# Autodesk Inventor assembly: Y_Axes
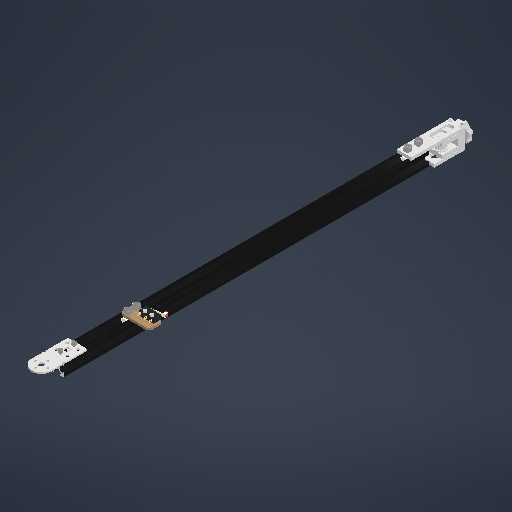
[picture p0: Inventor's stored thumbnail of the model, 512x512]
Saved by Autodesk Inventor 2027.1 (Build 311270010, 270A)
## iProperties
Created: 2026-10-02
Part Number: Y_Axes
Document SubType Name: Assembly
Designer: SDS Scholar
Author: SDS Scholar
## Documents named in this file (13)
- E:\Apps\AutodeskInventor\University\MCT333_Design_of_Mechatronics_Systems_1\CAD\cartesian_robot_workspace\Y_Axis.iam
- E:\Apps\AutodeskInventor\University\MCT333_Design_of_Mechatronics_Systems_1\CAD\off_the_shelf_components\AluminiumExtrusion\AluminiumExtrusion2020\Y_axis.ipt
- E:\Apps\AutodeskInventor\University\MCT333_Design_of_Mechatronics_Systems_1\CAD\off_the_shelf_components\GT2BeltTensioner\2020 Belt Tensioner G_K.ipt
- E:\Apps\AutodeskInventor\University\MCT333_Design_of_Mechatronics_Systems_1\CAD\off_the_shelf_components\T_nuts\Slider T-Nut for 2020 - M5.ipt
- C:\Users\SDS Scholar\Documents\Inventor\Content Center Files\R2027\en-US\SS-ISO 4762\ISO 4762 - M5 x 12SS-ISO.ipt
- E:\Apps\AutodeskInventor\University\MCT333_Design_of_Mechatronics_Systems_1\CAD\off_the_shelf_components\MotorMountPlate\motor holder bracket.ipt
- E:\Apps\AutodeskInventor\University\MCT333_Design_of_Mechatronics_Systems_1\CAD\off_the_shelf_components\T_nuts\Slider T-Nut for 2020 - M3.ipt
- C:\Users\SDS Scholar\Documents\Inventor\Content Center Files\R2027\en-US\ISO 4762(2)\ISO 4762 - M3 x 10ISO.ipt
- E:\Apps\AutodeskInventor\University\MCT333_Design_of_Mechatronics_Systems_1\CAD\cartesian_robot_workspace\LimitSwitchMountPlate.ipt
- C:\Users\SDS Scholar\Documents\Inventor\Content Center Files\R2027\en-US\SS-ISO 4762\ISO 4762 - M5 x 10SS-ISO.ipt
- E:\Apps\AutodeskInventor\University\MCT333_Design_of_Mechatronics_Systems_1\CAD\electronic_components\NO-NC Bump Switch\NO-NC Bump Switch.ipt
- C:\Users\SDS Scholar\Documents\Inventor\Content Center Files\R2027\en-US\DIN 7985 (H)\DIN 7985 (H) - M2.5x12-H.ipt
- C:\Users\SDS Scholar\Documents\Inventor\Content Center Files\R2027\en-US\ISO 4032(2)\ISO 4032 - M2.5 - ISO.ipt
## Components (21 placed, 12 different names)
1. Y_axis:1 — Mate:1, Mate:2, Mate:3, Mate:4, Mate:5, Mate:6, Mate:7, Mate:10, Mate:13, Mate:14, Flush:1, Mate:15, Mate:16, Mate:17, Mate:18, Mate:21, Mate:22, Mate:25, Flush:2, Mate:26, Mate:27, Mate:28, Mate:36, Mate:39, Mate:42, Mate:57
2. 2020 Belt Tensioner G_K:1 — Mate:8, Mate:11, Mate:14
3. SS ISO 4762 M5 x 12:1 — Mate:11, Mate:12, Mate:13
4. SS ISO 4762 M5 x 12:2 — Mate:8, Mate:9, Mate:10
5. Slider T-Nut for 2020 - M5:1 — Mate:4, Mate:5, Mate:9, Flush:1
6. Slider T-Nut for 2020 - M5:2 — Mate:6, Mate:7, Mate:12
7. motor holder bracket:1 — Mate:19, Mate:22, Mate:23, Mate:56
8. Slider T-Nut for 2020 - M3:1 — Mate:15, Mate:16, Mate:20
9. Slider T-Nut for 2020 - M3:2 — Mate:17, Mate:18, Mate:24, Flush:2
10. ISO 4762 M3 x 10:1 — Mate:23, Mate:24, Mate:25
11. ISO 4762 M3 x 10:2 — Mate:19, Mate:20, Mate:21
12. NO-NC Bump Switch:1 — Mate:45, Mate:47, Mate:48, Mate:49, Mate:51
13. LimitSwitchMountPlate:1 — Mate:36, Mate:37, Mate:40, Mate:46, Mate:48, Mate:50, Mate:54, Mate:55, Mate:56
14. Slider T-Nut for 2020 - M3:3 — Mate:28, Mate:41, Mate:57
15. Slider T-Nut for 2020 - M3:4 — Mate:26, Mate:27, Mate:38
16. SS ISO 4762 M5 x 10:1 — Mate:40, Mate:41, Mate:42
17. SS ISO 4762 M5 x 10:2 — Mate:37, Mate:38, Mate:39
18. DIN 7985 (H) M2.5x12-H:1 — Mate:45, Mate:46, Mate:47, Mate:52
19. DIN 7985 (H) M2.5x12-H:2 — Mate:49, Mate:50, Mate:51, Mate:53
20. ISO 4032 M2.5:1 — Mate:52, Mate:55
21. ISO 4032 M2.5:2 — Mate:53, Mate:54
## Relationships (50: Mate 48, Flush 2)
- Mate:1: Y_axis:1
- Mate:2: Y_axis:1
- Mate:3: Y_axis:1
- Mate:4: Y_axis:1 ↔ Slider T-Nut for 2020 - M5:1
- Mate:5: Y_axis:1 ↔ Slider T-Nut for 2020 - M5:1
- Mate:6: Y_axis:1 ↔ Slider T-Nut for 2020 - M5:2
- Mate:7: Y_axis:1 ↔ Slider T-Nut for 2020 - M5:2
- Mate:8: 2020 Belt Tensioner G_K:1 ↔ SS ISO 4762 M5 x 12:2
- Mate:9: SS ISO 4762 M5 x 12:2 ↔ Slider T-Nut for 2020 - M5:1
- Mate:10: Y_axis:1 ↔ SS ISO 4762 M5 x 12:2
- Mate:11: 2020 Belt Tensioner G_K:1 ↔ SS ISO 4762 M5 x 12:1
- Mate:12: SS ISO 4762 M5 x 12:1 ↔ Slider T-Nut for 2020 - M5:2
- Mate:13: Y_axis:1 ↔ SS ISO 4762 M5 x 12:1
- Mate:14: Y_axis:1 ↔ 2020 Belt Tensioner G_K:1
- Flush:1: Y_axis:1 ↔ Slider T-Nut for 2020 - M5:1
- Mate:15: Y_axis:1 ↔ Slider T-Nut for 2020 - M3:1
- Mate:16: Y_axis:1 ↔ Slider T-Nut for 2020 - M3:1
- Mate:17: Y_axis:1 ↔ Slider T-Nut for 2020 - M3:2
- Mate:18: Y_axis:1 ↔ Slider T-Nut for 2020 - M3:2
- Mate:19: motor holder bracket:1 ↔ ISO 4762 M3 x 10:2
- Mate:20: Slider T-Nut for 2020 - M3:1 ↔ ISO 4762 M3 x 10:2
- Mate:21: Y_axis:1 ↔ ISO 4762 M3 x 10:2
- Mate:22: Y_axis:1 ↔ motor holder bracket:1
- Mate:23: motor holder bracket:1 ↔ ISO 4762 M3 x 10:1
- Mate:24: Slider T-Nut for 2020 - M3:2 ↔ ISO 4762 M3 x 10:1
- Mate:25: Y_axis:1 ↔ ISO 4762 M3 x 10:1
- Flush:2: Y_axis:1 ↔ Slider T-Nut for 2020 - M3:2
- Mate:26: Y_axis:1 ↔ Slider T-Nut for 2020 - M3:4
- Mate:27: Y_axis:1 ↔ Slider T-Nut for 2020 - M3:4
- Mate:28: Y_axis:1 ↔ Slider T-Nut for 2020 - M3:3
- Mate:36: Y_axis:1 ↔ LimitSwitchMountPlate:1
- Mate:37: LimitSwitchMountPlate:1 ↔ SS ISO 4762 M5 x 10:2
- Mate:38: Slider T-Nut for 2020 - M3:4 ↔ SS ISO 4762 M5 x 10:2
- Mate:39: Y_axis:1 ↔ SS ISO 4762 M5 x 10:2
- Mate:40: LimitSwitchMountPlate:1 ↔ SS ISO 4762 M5 x 10:1
- Mate:41: Slider T-Nut for 2020 - M3:3 ↔ SS ISO 4762 M5 x 10:1
- Mate:42: Y_axis:1 ↔ SS ISO 4762 M5 x 10:1
- Mate:45: NO-NC Bump Switch:1 ↔ DIN 7985 (H) M2.5x12-H:1
- Mate:46: LimitSwitchMountPlate:1 ↔ DIN 7985 (H) M2.5x12-H:1
- Mate:47: NO-NC Bump Switch:1 ↔ DIN 7985 (H) M2.5x12-H:1
- Mate:48: NO-NC Bump Switch:1 ↔ LimitSwitchMountPlate:1
- Mate:49: NO-NC Bump Switch:1 ↔ DIN 7985 (H) M2.5x12-H:2
- Mate:50: LimitSwitchMountPlate:1 ↔ DIN 7985 (H) M2.5x12-H:2
- Mate:51: NO-NC Bump Switch:1 ↔ DIN 7985 (H) M2.5x12-H:2
- Mate:52: DIN 7985 (H) M2.5x12-H:1 ↔ ISO 4032 M2.5:1
- Mate:53: DIN 7985 (H) M2.5x12-H:2 ↔ ISO 4032 M2.5:2
- Mate:54: LimitSwitchMountPlate:1 ↔ ISO 4032 M2.5:2
- Mate:55: LimitSwitchMountPlate:1 ↔ ISO 4032 M2.5:1
- Mate:56 (65 mm): motor holder bracket:1 ↔ LimitSwitchMountPlate:1
- Mate:57: Y_axis:1 ↔ Slider T-Nut for 2020 - M3:3
